# Autodesk Inventor assembly: Steeping Complete Notification Contraption
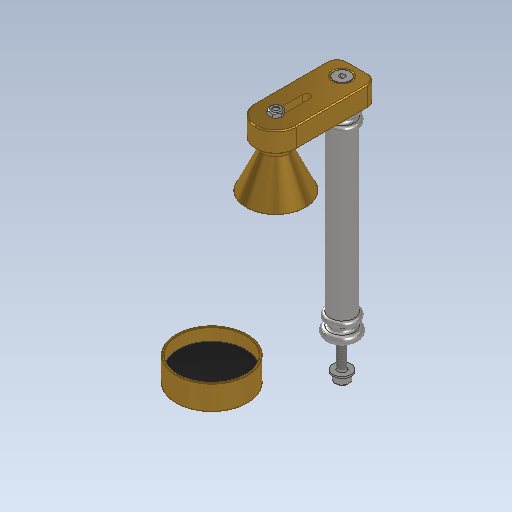
[picture p0: Inventor's stored thumbnail of the model, 512x512]
Saved by Autodesk Inventor 2021.1 (Build 251245010, 245A)
## iProperties
Created: 2025-09-16
Document SubType Name: Assembly
Designer: SD
Mass: 416.188 g
Surface Area: 229.329 cm^2
Volume: 50.2086 cm^3
Density: 8.28918 g/cm^3
Project: Automatic Tea Steeping mechanism
Part Number: Steeping Complete Notification Contraption
BOM-Mass: 0.41619
BOM-Area: 0.023
Author: SD
Title: Steeping Complete Notification Contraption
## Documents named in this file (13)
- S:\Future Scope 1\WIP\Client Category\Tom\02 Progressive Work\Steeping Complete Notification Contraption.iam
- S:\Future Scope 1\WIP\Client Category\Tom\02 Progressive Work\Bell Support Piller.ipt
- S:\Future Scope 1\WIP\Client Category\Tom\02 Progressive Work\Bell Support Beam.ipt
- S:\Future Scope 1\WIP\Client Category\Tom\02 Progressive Work\Bell.ipt
- S:\Future Scope 1\WIP\Client Category\Tom\02 Progressive Work\Hardware\Allen Key 4x25mm.ipt
- S:\Future Scope 1\WIP\Client Category\Tom\02 Progressive Work\Shallow Dish.ipt
- S:\Future Scope 1\WIP\Client Category\Tom\02 Progressive Work\Magnet.ipt
- S:\Future Scope 1\WIP\Client Category\Tom\02 Progressive Work\Foam Pad.ipt
- S:\Future Scope 1\WIP\Client Category\Tom\02 Progressive Work\4mm Washer.ipt
- S:\Future Scope 1\WIP\Client Category\Tom\02 Progressive Work\Hardware\M3 Hex Nut.ipt
- S:\Future Scope 1\WIP\Client Category\Tom\02 Progressive Work\Hardware\Allen Key 3x16mm.ipt
- S:\Future Scope 1\WIP\Client Category\Tom\02 Progressive Work\3mm Rubber Washer.ipt
- S:\Future Scope 1\WIP\Client Category\Tom\02 Progressive Work\Hardware\CSK Allen Key 4x20mm.ipt
## Components (13 placed, 12 different names)
1. Bell Support Beam:1 — Mate:17, Mate:31, Mate:33, Mate:34, Mate:35, Mate:36, Angle:1, Mate:40, Mate:42, Flush:2
2. Bell:1 — Mate:25, Mate:26, Mate:27, Mate:30
3. Allen Key 4x25mm:3 — Mate:23, Mate:24, Mate:41
4. Shallow Dish:1 — Mate:17, Mate:19, Mate:20, Mate:21, Mate:40, Flush:1
5. Magnet:1 — Mate:19, Mate:20, Mate:22
6. Foam Pad:1 — Mate:21, Mate:22
7. ISO 7089 4:1 — Mate:23, Mate:24, Mate:43
8. M3 Hex Nut:1 — Mate:29, Mate:30, Mate:34
9. ISO 4762 M3 x 5:1 — Mate:27, Mate:28, Mate:29, Mate:31, Mate:32
10. 3mm Rubber Washer:1 — Mate:25, Mate:26, Mate:28
11. M3 Hex Nut:2 — Mate:32, Mate:33
12. Bell Support Piller:1 — Mate:35, Mate:36, Mate:37, Mate:38, Mate:39, Flush:1, Mate:41, Mate:43
13. ISO 10642 M4x20:1 — Mate:42, Flush:2
## Relationships (29: Mate 26, Flush 2, Angle 1)
- Mate:17 (1.5 mm): Bell Support Beam:1 ↔ Shallow Dish:1
- Mate:19: Shallow Dish:1 ↔ Magnet:1
- Mate:20: Shallow Dish:1 ↔ Magnet:1
- Mate:21: Shallow Dish:1 ↔ Foam Pad:1
- Mate:22: Magnet:1 ↔ Foam Pad:1
- Mate:23: Allen Key 4x25mm:3 ↔ ISO 7089 4:1
- Mate:24: Allen Key 4x25mm:3 ↔ ISO 7089 4:1
- Mate:25: Bell:1 ↔ 3mm Rubber Washer:1
- Mate:26: Bell:1 ↔ 3mm Rubber Washer:1
- Mate:27: Bell:1 ↔ ISO 4762 M3 x 5:1
- Mate:28: ISO 4762 M3 x 5:1 ↔ 3mm Rubber Washer:1
- Mate:29: M3 Hex Nut:1 ↔ ISO 4762 M3 x 5:1
- Mate:30: Bell:1 ↔ M3 Hex Nut:1
- Mate:31: Bell Support Beam:1 ↔ ISO 4762 M3 x 5:1
- Mate:32: ISO 4762 M3 x 5:1 ↔ M3 Hex Nut:2
- Mate:33: Bell Support Beam:1 ↔ M3 Hex Nut:2
- Mate:34: Bell Support Beam:1 ↔ M3 Hex Nut:1
- Mate:35: Bell Support Beam:1 ↔ Bell Support Piller:1
- Mate:36: Bell Support Beam:1 ↔ Bell Support Piller:1
- Mate:37: Bell Support Piller:1
- Mate:38: Bell Support Piller:1
- Mate:39: Bell Support Piller:1
- Angle:1 (180 deg): Bell Support Beam:1
- Mate:40 (-60 mm): Bell Support Beam:1 ↔ Shallow Dish:1
- Flush:1: Shallow Dish:1 ↔ Bell Support Piller:1
- Mate:41: Allen Key 4x25mm:3 ↔ Bell Support Piller:1
- Mate:42: Bell Support Beam:1 ↔ ISO 10642 M4x20:1
- Flush:2: Bell Support Beam:1 ↔ ISO 10642 M4x20:1
- Mate:43 (14.7 mm): ISO 7089 4:1 ↔ Bell Support Piller:1
